# Autodesk Inventor assembly: Lampengehäuse
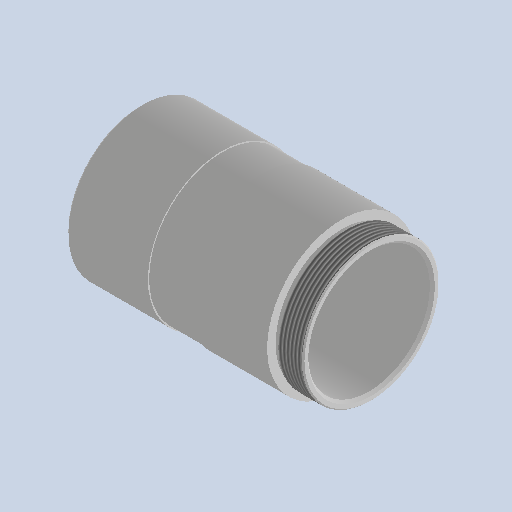
[picture p0: Inventor's stored thumbnail of the model, 512x512]
Saved by Autodesk Inventor 2022 (Build 260153000, 153)
## iProperties
Created: 2020-12-08
Part Number: Lampengehäuse
Document SubType Name: Assembly
Designer: g.schardt
Author: g.schardt
## Documents named in this file (3)
- Z:\g.schardt\Inventor\Tauchlampe\Lampengehäuse.iam
- Z:\g.schardt\Inventor\Tauchlampe\Glasscheibe.ipt
- Z:\g.schardt\Inventor\Tauchlampe\Lampengehäuse.ipt
## Components (2 placed, 2 different names)
1. Lampengehäuse:1 — Passend:1, Passend:2, Passend:3
2. Glasscheibe:1 — Passend:2, Passend:3
## Relationships (3: Mate 3)
- Passend:1 [Mate]: Lampengehäuse:1
- Passend:2 [Mate]: Lampengehäuse:1 ↔ Glasscheibe:1
- Passend:3 [Mate] (0.2 mm): Lampengehäuse:1 ↔ Glasscheibe:1
